# Autodesk Inventor assembly: rocket_asm
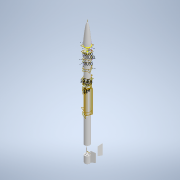
[picture p0: Inventor's stored thumbnail of the model, 180x180]
Saved by Autodesk Inventor 2020 (Build 240168000, 168)
## iProperties
Created: 2022-01-25
Part Number: rocket_asm
Document SubType Name: Assembly
Designer: sp
Author: sp
## Documents named in this file (13)
- C:\Users\sp\Documents\Rocket\rocket\CAD\rocket_asm.iam
- C:\Users\sp\Documents\Rocket\rocket\CAD\Segment_Engine.ipt
- C:\Users\sp\Documents\Rocket\rocket\CAD\Segment_mitte.ipt
- C:\Users\sp\Documents\Rocket\rocket\CAD\Segment_spitze.ipt
- C:\Users\sp\Documents\Rocket\rocket\CAD\Spitze.ipt
- C:\Users\sp\Documents\Rocket\rocket\CAD\Engine.ipt
- C:\Users\sp\Documents\Rocket\rocket\CAD\Leitwerk.ipt
- C:\Users\sp\Documents\Rocket\rocket\CAD\Back_holder.ipt
- C:\Users\sp\Documents\Rocket\rocket\CAD\Servo_Ku_asm.iam
- C:\Users\sp\Documents\Rocket\rocket\CAD\parachute_structure_asm.iam
- C:\Users\sp\Documents\Rocket\rocket\CAD\Elektro_asm.iam
- C:\Users\sp\Documents\Rocket\rocket\CAD\Ronde_Engine.ipt
- C:\Users\sp\Documents\Rocket\rocket\CAD\Deckel_Parachute_3.ipt
## Components (14 placed, 12 different names)
1. Segment_Engine:1 — Passend:1, Passend:2, Einfügen:3
2. Segment_mitte:1 — Passend:2, Passend:3, Einfügen:5, Passend:20, Passend:21
3. Segment_spitze:1 — Passend:3, Passend:6, Passend:19
4. Spitze:1 — Passend:1
5. Engine:1 — Passend:6, Passend:8, Fluchtend:1, Passend:9, Passend:10, Passend:11, Fluchtend:2, Passend:12, Passend:13, Fluchtend:3, Passend:15, Passend:16, Passend:18, Einfügen:4
6. Leitwerk:1 — Passend:8, Fluchtend:1, Passend:9
7. Leitwerk:2 — Passend:10, Passend:11, Fluchtend:2
8. Leitwerk:3 — Passend:12, Passend:13, Fluchtend:3
9. Back_holder:1 — Passend:15, Passend:16
10. Servo_Ku_asm:1 [sub-assembly] — Passend:20
11. parachute_structure_asm:1 [sub-assembly] — Einfügen:5, Passend:19
12. Elektro_asm:1 [sub-assembly] — Einfügen:3
13. Ronde_Engine:1 — Passend:18, Einfügen:4
14. Deckel_Parachute_3:1 — Passend:21
## Relationships (22: Mate 16, Flush 3, Insert 3)
- Passend:1 [Mate]: Segment_Engine:1 ↔ Spitze:1
- Passend:2 [Mate]: Segment_Engine:1 ↔ Segment_mitte:1
- Passend:3 [Mate]: Segment_mitte:1 ↔ Segment_spitze:1
- Passend:6 [Mate]: Segment_spitze:1 ↔ Engine:1
- Passend:8 [Mate]: Engine:1 ↔ Leitwerk:1
- Fluchtend:1 [Flush]: Engine:1 ↔ Leitwerk:1
- Passend:9 [Mate] (10.5 mm): Engine:1 ↔ Leitwerk:1
- Passend:10 [Mate]: Engine:1 ↔ Leitwerk:2
- Passend:11 [Mate]: Engine:1 ↔ Leitwerk:2
- Fluchtend:2 [Flush]: Engine:1 ↔ Leitwerk:2
- Passend:12 [Mate]: Engine:1 ↔ Leitwerk:3
- Passend:13 [Mate]: Engine:1 ↔ Leitwerk:3
- Fluchtend:3 [Flush]: Engine:1 ↔ Leitwerk:3
- Passend:15 [Mate]: Engine:1 ↔ Back_holder:1
- Passend:16 [Mate]: Engine:1 ↔ Back_holder:1
- Einfügen:3 [Insert]: Segment_Engine:1 ↔ Elektro_asm:1
- Passend:18 [Mate]: Engine:1 ↔ Ronde_Engine:1
- Einfügen:4 [Insert]: Engine:1 ↔ Ronde_Engine:1
- Einfügen:5 [Insert]: Segment_mitte:1 ↔ parachute_structure_asm:1
- Passend:19 [Mate]: Segment_spitze:1 ↔ parachute_structure_asm:1
- Passend:20 [Mate]: Segment_mitte:1 ↔ Servo_Ku_asm:1
- Passend:21 [Mate]: Segment_mitte:1 ↔ Deckel_Parachute_3:1
